# Autodesk Inventor assembly: Assembly
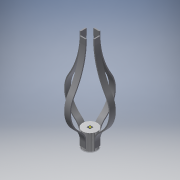
[picture p0: Inventor's stored thumbnail of the model, 180x180]
Saved by Autodesk Inventor 2016 (Build 200138000, 138)
## iProperties
Created: 2016-04-20
Part Number: Assembly
Document SubType Name: Assembly
Designer: Andres
Author: Andres
## Documents named in this file (7)
- \\Mac\Home\Documents\repositorios\BoreholeCamera\CAD_Probe\Assembly\Assembly.iam
- Z:\Documents\repositorios\BoreholeCamera\CAD_Probe\Enclosure\Parts\Enclosure.ipt
- Z:\Documents\repositorios\BoreholeCamera\CAD_Probe\Enclosure\Parts\Clamp.ipt
- Z:\Documents\repositorios\BoreholeCamera\CAD_Probe\Enclosure\Parts\ClampCover.ipt
- \\Mac\Home\Documents\repositorios\BoreholeCamera\CAD_Probe\Assembly\Assembly\Design Accelerator\Bolted Connection2.iam
- Z:\Documents\repositorios\BoreholeCamera\CAD_Probe\Enclosure\Parts\Cover.ipt
- Z:\Documents\repositorios\BoreholeCamera\CAD_Probe\Enclosure\Parts\8inch_Fin.ipt
## Components (9 placed, 6 different names)
1. Enclosure:1 — Rigid:1, Rigid:2, Rigid:3, Rigid:4, Rigid:5, Rigid:6, Rigid:7
2. Clamp:1 — Rigid:1
3. ClampCover:1 — Rigid:2, Mate:1, Mate:2
4. Bolted Connection:1 [sub-assembly] — Mate:1, Mate:2
5. Cover:1 — Rigid:3
6. 8inch_Fin:1 — Rigid:4
7. 8inch_Fin:2 — Rigid:5
8. 8inch_Fin:3 — Rigid:6
9. 8inch_Fin:4 — Rigid:7
## Relationships (9: WeldJoint 7, Mate 2)
- Rigid:1 [WeldJoint]: Enclosure:1 ↔ Clamp:1
- Rigid:2 [WeldJoint]: Enclosure:1 ↔ ClampCover:1
- Mate:1: ClampCover:1 ↔ Bolted Connection:1
- Mate:2: ClampCover:1 ↔ Bolted Connection:1
- Rigid:3 [WeldJoint]: Enclosure:1 ↔ Cover:1
- Rigid:4 [WeldJoint]: Enclosure:1 ↔ 8inch_Fin:1
- Rigid:5 [WeldJoint]: Enclosure:1 ↔ 8inch_Fin:2
- Rigid:6 [WeldJoint]: Enclosure:1 ↔ 8inch_Fin:3
- Rigid:7 [WeldJoint]: Enclosure:1 ↔ 8inch_Fin:4
